# Autodesk Inventor assembly: Lagerhalterung_ohne_Platte
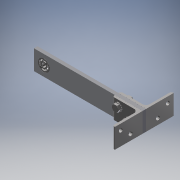
[picture p0: Inventor's stored thumbnail of the model, 180x180]
Saved by Autodesk Inventor 2018 (Build 220112000, 112)
## iProperties
Created: 2018-01-29
Part Number: Lagerhalterung_ohne_Platte
Material: Generisch
Document SubType Name: Assembly
Designer: Julian
Author: Julian
## Documents named in this file (7)
- C:\Users\Julian\Desktop\Schule\5AHME\Diplomarbeit\Git\fuettr_prototype\Mechanical\Inventorskizzen\Lagerhalterung_ohne_Platte.iam
- C:\Users\Julian\Desktop\Schule\5AHME\Diplomarbeit\Git\fuettr_prototype\Mechanical\Inventorskizzen\ISO 657-1 - L70x70x6-50.ipt
- C:\Users\Julian\Documents\Inventor\Content Center Files\R2018\de-DE\ISO 7090\ISO 7090 - 10 - 140 HV(1).ipt
- C:\Users\Julian\Documents\Inventor\Content Center Files\R2018\de-DE\ISO 4017(1)\ISO 4017 - M10 x 35 - ISO.ipt
- C:\Users\Julian\Documents\Inventor\Content Center Files\R2018\de-DE\ISO 4032(2)\ISO 4032 - M10 - ISO.ipt
- C:\Users\Julian\Documents\Inventor\Content Center Files\R2018\de-DE\DIN 625 SKF(4)\DIN 625 SKF - SKF 6200-2Z.ipt
- C:\Users\Julian\Desktop\Schule\5AHME\Diplomarbeit\Git\fuettr_prototype\Mechanical\Inventorskizzen\Lagerstuetze_kurz.ipt
## Components (12 placed, 6 different names)
1. ISO 657-1 - L70x70x6-50:1 — Starr:1, Passend:1, Passend:2, Starr:3
2. ISO 657-1 - L70x70x6-50:2 — Starr:2, Starr:4, Starr:5
3. Lagerstuetze_kurz:1 — Starr:1, Starr:2, Starr:18
4. ISO 7090 10 - 140 HV:1 — Passend:1, Passend:2, Starr:6
5. ISO 7090 10 - 140 HV:2 — Starr:3, Starr:7
6. ISO 7090 10 - 140 HV:3 — Starr:4, Starr:8
7. ISO 7090 10 - 140 HV:4 — Starr:5, Drehbar:1
8. ISO 4017 M10 x 35:1 — Starr:7
9. ISO 4017 M10 x 35:2 — Starr:6
10. ISO 4032 M10:1 — Starr:8
11. ISO 4032 M10:2 — Drehbar:1
12. DIN 625 SKF- beidseitig abgedeckt SKF 6200-2Z:1 — Starr:18
## Relationships (12: WeldJoint 9, Mate 2, RevoluteJoint 1)
- Starr:1 [WeldJoint]: ISO 657-1 - L70x70x6-50:1 ↔ Lagerstuetze_kurz:1
- Starr:2 [WeldJoint]: ISO 657-1 - L70x70x6-50:2 ↔ Lagerstuetze_kurz:1
- Passend:1 [Mate]: ISO 657-1 - L70x70x6-50:1 ↔ ISO 7090 10 - 140 HV:1
- Passend:2 [Mate]: ISO 657-1 - L70x70x6-50:1 ↔ ISO 7090 10 - 140 HV:1
- Starr:3 [WeldJoint]: ISO 657-1 - L70x70x6-50:1 ↔ ISO 7090 10 - 140 HV:2
- Starr:4 [WeldJoint]: ISO 657-1 - L70x70x6-50:2 ↔ ISO 7090 10 - 140 HV:3
- Starr:5 [WeldJoint]: ISO 657-1 - L70x70x6-50:2 ↔ ISO 7090 10 - 140 HV:4
- Starr:6 [WeldJoint]: ISO 7090 10 - 140 HV:1 ↔ ISO 4017 M10 x 35:2
- Starr:7 [WeldJoint]: ISO 7090 10 - 140 HV:2 ↔ ISO 4017 M10 x 35:1
- Starr:8 [WeldJoint]: ISO 7090 10 - 140 HV:3 ↔ ISO 4032 M10:1
- Drehbar:1 [RevoluteJoint]: ISO 7090 10 - 140 HV:4 ↔ ISO 4032 M10:2
- Starr:18 [WeldJoint]: Lagerstuetze_kurz:1 ↔ DIN 625 SKF- beidseitig abgedeckt SKF 6200-2Z:1
